# Autodesk Inventor assembly: Ari Tsugi
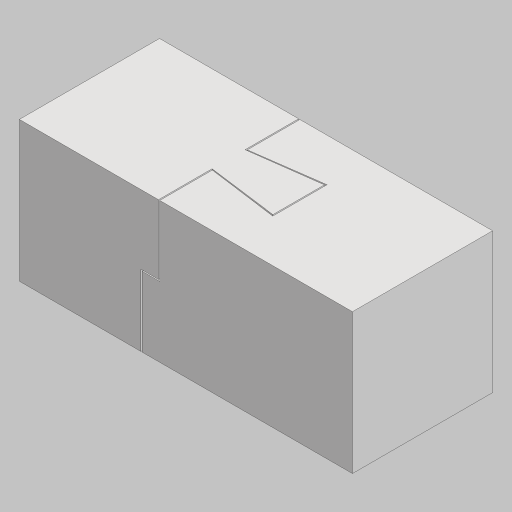
[picture p0: Inventor's stored thumbnail of the model, 512x512]
Saved by Autodesk Inventor 2023 (Build 270158000, 158)
## iProperties
Created: 2026-02-22
Part Number: Ari Tsugi
Document SubType Name: Assembly
Designer: MARTIN MAESTRE
Author: MARTIN MAESTRE
## Documents named in this file (3)
- C:\Users\MARTIN MAESTRE\OneDrive - Universidad de los Andes\POSTGRADO\202610\MAESTRIA\PROBLEMA ESPECIAL\Tolerancias\0.30mm\Fig2_0.30\Ari Tsugi_0.30.iam
- C:\Users\MARTIN MAESTRE\OneDrive - Universidad de los Andes\POSTGRADO\202610\MAESTRIA\PROBLEMA ESPECIAL\Tolerancias\0.30mm\Fig2_0.30\Macho.ipt
- C:\Users\MARTIN MAESTRE\OneDrive - Universidad de los Andes\POSTGRADO\202610\MAESTRIA\PROBLEMA ESPECIAL\Tolerancias\0.30mm\Fig2_0.30\Hembra.ipt
## Components (2 placed, 2 different names)
1. Macho:1 — Nivelación:1, Coincidencia:2, Nivelación:2
2. Hembra:1 — Coincidencia:3, Nivelación:2
## Relationships (4: Flush 2, Mate 2)
- Nivelación:1 [Flush]: Macho:1
- Coincidencia:2 [Mate]: Macho:1
- Coincidencia:3 [Mate]: Hembra:1
- Nivelación:2 [Flush]: Macho:1 ↔ Hembra:1
